# Autodesk Inventor assembly: Ensamblaje_portaplatos
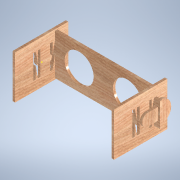
[picture p0: Inventor's stored thumbnail of the model, 180x180]
Saved by Autodesk Inventor 2022 (Build 260153000, 153)
## iProperties
Created: 2023-02-12
Part Number: Ensamblaje_portaplatos
Document SubType Name: Assembly
Designer: USUARIO
Author: USUARIO
## Documents named in this file (4)
- C:\Users\USUARIO\Documents\Academico\2023-I\APM\Modelo comedero\Ensamblaje_portaplatos.iam
- C:\Users\USUARIO\Documents\Academico\2023-I\APM\Modelo comedero\Parte A-B.ipt
- C:\Users\USUARIO\Documents\Academico\2023-I\APM\Modelo comedero\Parte C.ipt
- C:\Users\USUARIO\Documents\Academico\2023-I\APM\Modelo comedero\Parte D.ipt
## Components (5 placed, 3 different names)
1. Parte A-B:1 — Coincidencia:1, Coincidencia:2, Coincidencia:3
2. Parte A-B:2 — Coincidencia:4, Coincidencia:5, Coincidencia:6
3. Parte C:1 — Coincidencia:1, Coincidencia:2, Coincidencia:3, Coincidencia:4, Coincidencia:5, Coincidencia:6, Coincidencia:7, Coincidencia:8, Coincidencia:9, Coincidencia:10
4. Parte D:1 — Coincidencia:9, Coincidencia:10
5. Parte D:2 — Coincidencia:7, Coincidencia:8
## Relationships (10: Mate 10)
- Coincidencia:1 [Mate]: Parte A-B:1 ↔ Parte C:1
- Coincidencia:2 [Mate]: Parte A-B:1 ↔ Parte C:1
- Coincidencia:3 [Mate]: Parte A-B:1 ↔ Parte C:1
- Coincidencia:4 [Mate]: Parte A-B:2 ↔ Parte C:1
- Coincidencia:5 [Mate]: Parte A-B:2 ↔ Parte C:1
- Coincidencia:6 [Mate]: Parte A-B:2 ↔ Parte C:1
- Coincidencia:7 [Mate]: Parte C:1 ↔ Parte D:2
- Coincidencia:8 [Mate]: Parte C:1 ↔ Parte D:2
- Coincidencia:9 [Mate]: Parte C:1 ↔ Parte D:1
- Coincidencia:10 [Mate]: Parte C:1 ↔ Parte D:1
